# Autodesk Inventor assembly: assembly extruder
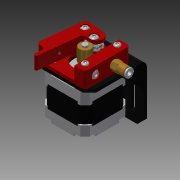
[picture p0: Inventor's stored thumbnail of the model, 180x180]
Saved by Autodesk Inventor 2015 (Build 190159000, 159)
## iProperties
Created: 2015-02-19
Part Number: assembly extruder
Document SubType Name: Assembly
Designer: Noa Izumi
Author: Noa Izumi
## Documents named in this file (13)
- E:\3D_Designs\Inventor\3D Printer\TinyBoy-master\src\assembly extruder.iam
- E:\3D_Designs\Inventor\3D Printer\TinyBoy-master\src\stepper_42.iam
- E:\3D_Designs\Inventor\3D Printer\TinyBoy-master\src\stepper_mount_42.ipt
- E:\3D_Designs\Inventor\3D Printer\TinyBoy-master\src\extruder_base.ipt
- E:\3D_Designs\Inventor\3D Printer\TinyBoy-master\src\screw_M3_22_hex.ipt
- E:\3D_Designs\Inventor\3D Printer\TinyBoy-master\src\screw_M3_10_hex.ipt
- E:\3D_Designs\Inventor\3D Printer\TinyBoy-master\src\screw_M4_10_hex.ipt
- E:\3D_Designs\Inventor\3D Printer\TinyBoy-master\src\pc4_m6.ipt
- E:\3D_Designs\Inventor\3D Printer\TinyBoy-master\src\extruder_gear.ipt
- E:\3D_Designs\Inventor\3D Printer\TinyBoy-master\src\extruder_lever.ipt
- E:\3D_Designs\Inventor\3D Printer\TinyBoy-master\src\washer_M3.ipt
- E:\3D_Designs\Inventor\3D Printer\TinyBoy-master\src\bearing_604uu.ipt
- E:\3D_Designs\Inventor\3D Printer\TinyBoy-master\src\washer_M4.ipt
## Components (16 placed, 12 different names)
1. stepper_42:1 [sub-assembly] — 插入:1, 插入:2, 插入:10
2. stepper_mount_42:1 — 插入:1, 插入:2, 插入:3, 插入:4
3. extruder_base:1 — 插入:3, 插入:4, 插入:5, 插入:6, 插入:7, 插入:8, 插入:9, 角度:1, Mate:1, Cylindrical:1
4. screw_M3_22_hex:1 — 插入:6
5. screw_M3_22_hex:2 — 插入:5
6. screw_M3_10_hex:1 — 插入:8
7. screw_M4_10_hex:1 — 插入:7
8. pc4_m6:1 — 插入:9, 角度:1
9. extruder_gear:1 — 插入:10
10. extruder_lever:1 — 插入:16, 插入:17, Mate:1, Cylindrical:1, Mate:2, Mate:3
11. washer_M3:1 — Insert:18, Mate:2
12. screw_M3_22_hex:3 — Insert:18, Mate:3
13. bearing_604uu:1 — 插入:14, 插入:15
14. screw_M4_10_hex:2 — 插入:17
15. washer_M4:1 — 插入:14, 插入:16
16. washer_M4:2 — 插入:15
## Relationships (20: Insert 15, Mate 3, Angle 1, CylindricalJoint 1)
- 插入:1 [Insert] (0.5 mm): stepper_42:1 ↔ stepper_mount_42:1
- 插入:2 [Insert]: stepper_42:1 ↔ stepper_mount_42:1
- 插入:3 [Insert]: stepper_mount_42:1 ↔ extruder_base:1
- 插入:4 [Insert]: stepper_mount_42:1 ↔ extruder_base:1
- 插入:5 [Insert]: extruder_base:1 ↔ screw_M3_22_hex:2
- 插入:6 [Insert]: extruder_base:1 ↔ screw_M3_22_hex:1
- 插入:7 [Insert]: extruder_base:1 ↔ screw_M4_10_hex:1
- 插入:8 [Insert]: extruder_base:1 ↔ screw_M3_10_hex:1
- 插入:9 [Insert]: extruder_base:1 ↔ pc4_m6:1
- 角度:1 [Angle] (0 deg): extruder_base:1 ↔ pc4_m6:1
- 插入:10 [Insert] (1.5 mm): stepper_42:1 ↔ extruder_gear:1
- 插入:14 [Insert]: bearing_604uu:1 ↔ washer_M4:1
- 插入:15 [Insert]: bearing_604uu:1 ↔ washer_M4:2
- 插入:16 [Insert]: extruder_lever:1 ↔ washer_M4:1
- 插入:17 [Insert]: extruder_lever:1 ↔ screw_M4_10_hex:2
- Mate:1: extruder_base:1 ↔ extruder_lever:1
- Cylindrical:1: extruder_base:1 ↔ extruder_lever:1
- Insert:18: washer_M3:1 ↔ screw_M3_22_hex:3
- Mate:2: extruder_lever:1 ↔ washer_M3:1
- Mate:3: extruder_lever:1 ↔ screw_M3_22_hex:3
